# Autodesk Inventor assembly: 足全体
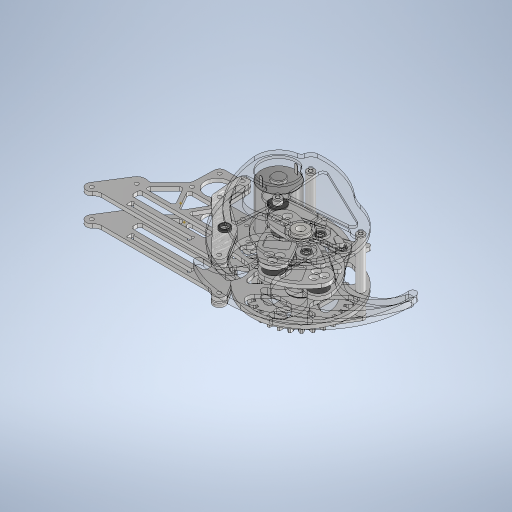
[picture p0: Inventor's stored thumbnail of the model, 512x512]
Saved by Autodesk Inventor 2023 (Build 270158000, 158)
## iProperties
Created: 2022-01-30
Part Number: 足全体
Document SubType Name: Assembly
Designer: acps
Author: acps
## Documents named in this file (7)
- C:\Users\acps\Documents\srdc\srdc_ksh\脚\足全体.iam
- C:\Users\acps\Documents\srdc\srdc_ksh\脚\アーノン.ipt
- C:\Users\acps\Documents\srdc\srdc_ksh\脚\足ユニット.iam
- C:\Users\acps\Documents\srdc\srdc_ksh\脚\中間ユニット内.ipt
- C:\Users\acps\Documents\srdc\srdc_ksh\オイレス\w5f6-12a.ipt
- C:\Users\acps\Documents\srdc\srdc_ksh\スペーサ\l4.ipt
- C:\Users\acps\Documents\srdc\srdc_ksh\スペーサ\l19.ipt
## Components (10 placed, 6 different names)
1. 足ユニット:1 [sub-assembly] — Insert:8
2. アーノン:1 — Mate:6, Insert:3, Mate:8
3. アーノン:2 — Mate:5, Insert:10
4. 中間ユニット内:1 — Mate:8, Insert:13
5. 中間ユニット内:2 — Mate:5, Mate:12, Insert:11, Insert:12
6. w5f6-12a:1 — Mate:9, Mate:12, Insert:9, Insert:10, Insert:11
7. w5f6-12a:2 — Mate:6, Insert:3, Mate:10, Insert:6
8. l4:1 — Mate:10, Insert:6
9. l4:2 — Mate:9, Insert:9
10. l19:1 — Insert:8, Insert:12, Insert:13
## Relationships (14: Insert 8, Mate 6)
- Mate:5: アーノン:2 ↔ 中間ユニット内:2
- Mate:6: アーノン:1 ↔ w5f6-12a:2
- Insert:3: アーノン:1 ↔ w5f6-12a:2
- Mate:8: アーノン:1 ↔ 中間ユニット内:1
- Mate:9: w5f6-12a:1 ↔ l4:2
- Mate:10: w5f6-12a:2 ↔ l4:1
- Insert:6: w5f6-12a:2 ↔ l4:1
- Mate:12: 中間ユニット内:2 ↔ w5f6-12a:1
- Insert:8: 足ユニット:1 ↔ l19:1
- Insert:9: w5f6-12a:1 ↔ l4:2
- Insert:10: アーノン:2 ↔ w5f6-12a:1
- Insert:11: 中間ユニット内:2 ↔ w5f6-12a:1
- Insert:12 (0.1 mm): 中間ユニット内:2 ↔ l19:1
- Insert:13 (0.1 mm): 中間ユニット内:1 ↔ l19:1
